# Autodesk Inventor assembly: FullSailCapstan-ver1-1111-2021
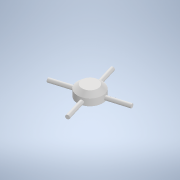
[picture p0: Inventor's stored thumbnail of the model, 180x180]
Saved by Autodesk Inventor 2021 (Build 250183000, 183)
## iProperties
Created: 2021-03-03
Part Number: FullSailCapstan-ver1-1111-2021
Document SubType Name: Assembly
Designer: CMurray
Author: CMurray
## Documents named in this file (3)
- F:\PHRC CADD 2021\2021 Game Design Challenge\Crow's Nest\Parts\Capstan\FullSailCapstan-ver1-1111-2021.iam
- F:\PHRC CADD 2021\2021 Game Design Challenge\Crow's Nest\Parts\Capstan\UpperSailCapMid-ver1-1111-2021.ipt
- F:\PHRC CADD 2021\2021 Game Design Challenge\Crow's Nest\Parts\Capstan\UpperSailCapTop-ver1-1111-2021.ipt
## Components (2 placed, 2 different names)
1. UpperSailCapMid-ver1-1111-2021:1 — Mate:1, Rotational:1
2. UpperSailCapTop-ver1-1111-2021:1 — Mate:1, Rotational:1
## Relationships (2: Mate 1, RevoluteJoint 1)
- Mate:1: UpperSailCapMid-ver1-1111-2021:1 ↔ UpperSailCapTop-ver1-1111-2021:1
- Rotational:1 [RevoluteJoint]: UpperSailCapMid-ver1-1111-2021:1 ↔ UpperSailCapTop-ver1-1111-2021:1
